# Autodesk Inventor assembly: BASE_002
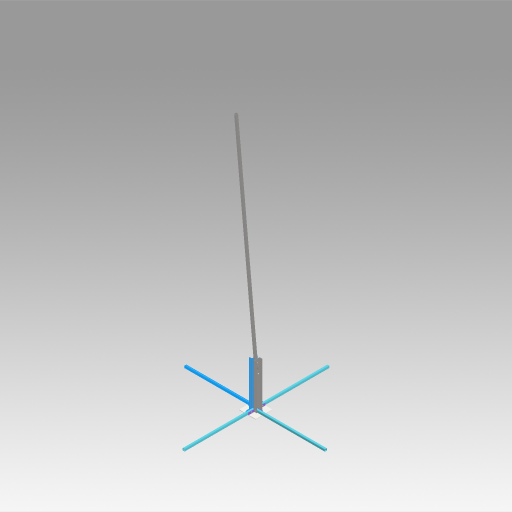
[picture p0: Inventor's stored thumbnail of the model, 512x512]
Saved by Autodesk Inventor 2023 (Build 270158000, 158)
## iProperties
Created: 2025-04-08
Part Number: BASE_002
Document SubType Name: Assembly
Designer: NELLY NDUNG'U
Author: NELLY NDUNG'U
## Documents named in this file (14)
- N:\NAKUJA\CAD FILES\AIRFRAME\LP002\BASE_002.iam
- N:\NAKUJA\CAD FILES\AIRFRAME\LP002\U_SECTION.iam
- N:\NAKUJA\CAD FILES\AIRFRAME\LP002\BASE PLATE.ipt
- N:\NAKUJA\CAD FILES\AIRFRAME\LP002\LEG.iam
- N:\NAKUJA\CAD FILES\AIRFRAME\LP002\RAIL_SUPPORT.iam
- C:\Users\User\Documents\Inventor\Content Center Files\R2023\en-US\ANSI B18.2.3.5M\ANSI B18.2.3.5M - M16 x 2 x 70.ipt
- C:\Users\User\Documents\Inventor\Content Center Files\R2023\en-US\ANSI B 18.2.4.1 M(1)\ANSI B 18.2.4.1 M - M14 x 2Style 1.ipt
- C:\Users\User\Documents\Inventor\Content Center Files\R2023\en-US\ANSI B 18.2.4.1 M(1)\ANSI B 18.2.4.1 M - M16 x 2Style 1.ipt
- N:\NAKUJA\CAD FILES\AIRFRAME\LP002\BASE_002\AIP\FEA\f120kkalc.fins
- N:\NAKUJA\CAD FILES\AIRFRAME\LP002\BASE_002\AIP\FEA\f120kkam8.fsat
- N:\NAKUJA\CAD FILES\AIRFRAME\LP002\BASE_002\AIP\FEA\f120kkam8.ftes
- N:\NAKUJA\CAD FILES\AIRFRAME\LP002\BASE_002\AIP\FEA\f120kkam8.fwiz
- N:\NAKUJA\CAD FILES\AIRFRAME\LP002\BASE_002\AIP\FEA\f120kkbfk.fmsh
- N:\NAKUJA\CAD FILES\AIRFRAME\LP002\BASE_002\AIP\FEA\f120kkbfl.fres
## Components (20 placed, 7 different names)
1. U_SECTION:1 [sub-assembly] — Mate:1, Mate:2, Mate:3, Mate:6, Flush:2, Flush:3, Insert:8, Insert:9, Insert:10, Insert:11, Insert:13, Insert:14, Insert:15
2. U_SECTION:2 [sub-assembly] — Mate:4, Flush:1, Mate:5, Mate:7, Mate:9, Mate:10, Angle:1, Mate:11, Mate:12, Mate:13, Insert:5, Insert:6, Insert:7, Insert:12, Insert:16, Insert:17, Insert:18
3. BASE PLATE:1 — Mate:1, Mate:2, Mate:3, Mate:4, Flush:1, Mate:5
4. LEG:1 [sub-assembly] — Mate:6, Mate:7, Flush:2
5. LEG:2 [sub-assembly] — Flush:3, Mate:9, Mate:10
6. RAIL_SUPPORT:1 [sub-assembly] — Angle:1, Mate:11, Mate:12, Mate:13
7. Hex Bolt - Metric M16 x 2 x 70:1 — Insert:6
8. Hex Bolt - Metric M16 x 2 x 70:2 — Insert:7
9. Hex Bolt - Metric M16 x 2 x 70:3 — Insert:5
10. Hex Bolt - Metric M16 x 2 x 70:4 — Insert:8
11. Hex Nut Metric M14 x 2:1 — Insert:9
12. Hex Nut Metric M14 x 2:2 — Insert:10
13. Hex Nut Metric M14 x 2:3 — Insert:11
14. Hex Nut Metric M14 x 2:4 — Insert:12
15. Hex Bolt - Metric M16 x 2 x 70:5 — Insert:13
16. Hex Bolt - Metric M16 x 2 x 70:6 — Insert:14
17. Hex Bolt - Metric M16 x 2 x 70:7 — Insert:15
18. Hex Nut Metric M16 x 2:1 — Insert:16
19. Hex Nut Metric M16 x 2:2 — Insert:17
20. Hex Nut Metric M16 x 2:3 — Insert:18
## Relationships (30: Insert 14, Mate 12, Flush 3, Angle 1)
- Mate:1: U_SECTION:1 ↔ BASE PLATE:1
- Mate:2 (-130 mm): U_SECTION:1 ↔ BASE PLATE:1
- Mate:3 (-100 mm): U_SECTION:1 ↔ BASE PLATE:1
- Mate:4: U_SECTION:2 ↔ BASE PLATE:1
- Flush:1 (100 mm): U_SECTION:2 ↔ BASE PLATE:1
- Mate:5 (-130 mm): U_SECTION:2 ↔ BASE PLATE:1
- Mate:6: U_SECTION:1 ↔ LEG:1
- Mate:7 (5 mm): U_SECTION:2 ↔ LEG:1
- Flush:2: U_SECTION:1 ↔ LEG:1
- Flush:3: U_SECTION:1 ↔ LEG:2
- Mate:9: U_SECTION:2 ↔ LEG:2
- Mate:10 (-5 mm): U_SECTION:2 ↔ LEG:2
- Angle:1 (85 deg): U_SECTION:2 ↔ RAIL_SUPPORT:1
- Mate:11 (300 mm): U_SECTION:2 ↔ RAIL_SUPPORT:1
- Mate:12: U_SECTION:2 ↔ RAIL_SUPPORT:1
- Mate:13 (-8 mm): U_SECTION:2 ↔ RAIL_SUPPORT:1
- Insert:5: U_SECTION:2 ↔ Hex Bolt - Metric M16 x 2 x 70:3
- Insert:6: U_SECTION:2 ↔ Hex Bolt - Metric M16 x 2 x 70:1
- Insert:7: U_SECTION:2 ↔ Hex Bolt - Metric M16 x 2 x 70:2
- Insert:8: U_SECTION:1 ↔ Hex Bolt - Metric M16 x 2 x 70:4
- Insert:9: U_SECTION:1 ↔ Hex Nut Metric M14 x 2:1
- Insert:10: U_SECTION:1 ↔ Hex Nut Metric M14 x 2:2
- Insert:11: U_SECTION:1 ↔ Hex Nut Metric M14 x 2:3
- Insert:12: U_SECTION:2 ↔ Hex Nut Metric M14 x 2:4
- Insert:13: U_SECTION:1 ↔ Hex Bolt - Metric M16 x 2 x 70:5
- Insert:14: U_SECTION:1 ↔ Hex Bolt - Metric M16 x 2 x 70:6
- Insert:15: U_SECTION:1 ↔ Hex Bolt - Metric M16 x 2 x 70:7
- Insert:16: U_SECTION:2 ↔ Hex Nut Metric M16 x 2:1
- Insert:17: U_SECTION:2 ↔ Hex Nut Metric M16 x 2:2
- Insert:18: U_SECTION:2 ↔ Hex Nut Metric M16 x 2:3
## Named parameters: sa_0 = 52300
note: some values were not read from the file. Shown as the stored number, unit unknown: "sa_0".
